# Autodesk Inventor assembly: recuperation
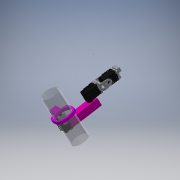
[picture p0: Inventor's stored thumbnail of the model, 180x180]
Saved by Autodesk Inventor 2017 (Build 210142000, 142)
## iProperties
Created: 2018-03-31
Part Number: recuperation
Document SubType Name: Assembly
Designer: franc
Mass: 403.773 g
Surface Area: 1652.88 cm^2
Volume: 403.773 cm^3
Density: 1 g/cm^3
Author: franc
## Documents named in this file (8)
- C:\Users\franc\Desktop\EsialRobotik\Mecanique\2018\robot\traitement-eau\recuperation.iam
- C:\Users\franc\Desktop\EsialRobotik\Mecanique\2018\robot\traitement-eau\cylindre-stockage.ipt
- C:\Users\franc\Desktop\EsialRobotik\Mecanique\composants\AX12\AX12.iam
- C:\Users\franc\Desktop\EsialRobotik\Mecanique\composants\AX12\F3.ipt
- C:\Users\franc\Desktop\EsialRobotik\Mecanique\composants\AX12\F2.ipt
- C:\Users\franc\Desktop\EsialRobotik\Mecanique\2018\robot\traitement-eau\rotation-recuperation.ipt
- C:\Users\franc\Desktop\EsialRobotik\Mecanique\2018\robot\traitement-eau\bras.ipt
- C:\Users\franc\Desktop\EsialRobotik\Mecanique\2018\robot\traitement-eau\fixation-bras.ipt
## Components (10 placed, 7 different names)
1. cylindre-stockage:1 — Tangente:9, Affleurement:3, Placage:22
2. F2:1 — Tangente:9, Affleurement:3, Placage:14, Affleurement:5, Placage:25, Placage:26, Placage:27
3. rotation-recuperation:1 — Placage:14, Affleurement:5, Placage:22
4. bras:1 — Placage:28, Placage:29, Placage:30, Placage:31, Placage:32, Placage:33
5. AX12:2 [sub-assembly] — Placage:31, Placage:32, Placage:33, Placage:37, Placage:38, Placage:39
6. AX12:3 [sub-assembly] — Placage:25, Placage:26, Placage:27, Placage:28, Placage:29, Placage:30
7. AX12:4 [sub-assembly] — Placage:34, Placage:35, Placage:36, Placage:43, Placage:44, Placage:45
8. F2:2 — Placage:34, Placage:35, Placage:36, Placage:40, Placage:41, Placage:42
9. F3:2 — Placage:37, Placage:38, Placage:39, Placage:40, Placage:41, Placage:42
10. fixation-bras:1 — Placage:43, Placage:44, Placage:45
## Relationships (26: Mate 23, Flush 2, Tangent 1)
- Tangente:9 (1 mm): cylindre-stockage:1 ↔ F2:1
- Affleurement:3 [Flush] (87.5 mm): cylindre-stockage:1 ↔ F2:1
- Placage:14 [Mate]: F2:1 ↔ rotation-recuperation:1
- Affleurement:5 [Flush]: F2:1 ↔ rotation-recuperation:1
- Placage:22 [Mate]: cylindre-stockage:1 ↔ rotation-recuperation:1
- Placage:25 [Mate]: F2:1 ↔ AX12:3
- Placage:26 [Mate]: F2:1 ↔ AX12:3
- Placage:27 [Mate]: F2:1 ↔ AX12:3
- Placage:28 [Mate]: bras:1 ↔ AX12:3
- Placage:29 [Mate]: bras:1 ↔ AX12:3
- Placage:30 [Mate]: bras:1 ↔ AX12:3
- Placage:31 [Mate]: bras:1 ↔ AX12:2
- Placage:32 [Mate]: bras:1 ↔ AX12:2
- Placage:33 [Mate]: bras:1 ↔ AX12:2
- Placage:34 [Mate]: AX12:4 ↔ F2:2
- Placage:35 [Mate]: AX12:4 ↔ F2:2
- Placage:36 [Mate]: AX12:4 ↔ F2:2
- Placage:37 [Mate]: AX12:2 ↔ F3:2
- Placage:38 [Mate]: AX12:2 ↔ F3:2
- Placage:39 [Mate]: AX12:2 ↔ F3:2
- Placage:40 [Mate]: F2:2 ↔ F3:2
- Placage:41 [Mate]: F2:2 ↔ F3:2
- Placage:42 [Mate]: F2:2 ↔ F3:2
- Placage:43 [Mate]: AX12:4 ↔ fixation-bras:1
- Placage:44 [Mate]: AX12:4 ↔ fixation-bras:1
- Placage:45 [Mate]: AX12:4 ↔ fixation-bras:1
